# Autodesk Inventor assembly: link9_SubAssembly.ipt
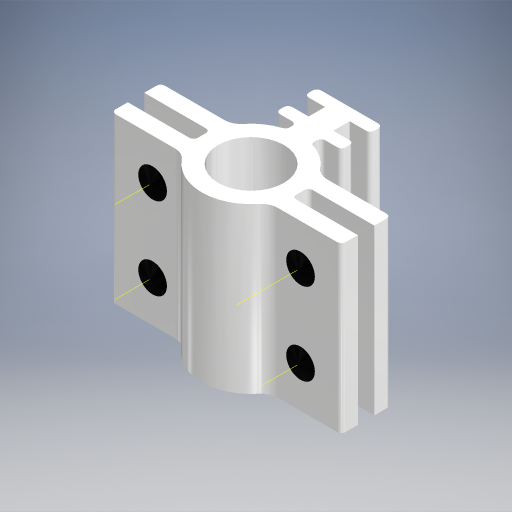
[picture p0: Inventor's stored thumbnail of the model, 512x512]
Saved by Autodesk Inventor 2024.1 (Build 281209000, 209)
## iProperties
Created: 2023-11-11
Part Number: link9_SubAssembly.ipt
Document SubType Name: Assembly
Designer: Camilo
Mass: 8.97147 g
Surface Area: 38.2594 cm^2
Volume: 3.32277 cm^3
Density: 2.7 g/cm^3
Author: Camilo
## Documents named in this file (3)
- D:\Documentos\MEGA\Universidad\2023-2\DinamicaComputacionalDeSistemasMulticuerpo\DinamicaComputacionalSistemasMulticuerpo\Proyecto\CAD\3D\link5_SubAssembly.iam
- D:\Documentos\MEGA\Universidad\2023-2\DinamicaComputacionalDeSistemasMulticuerpo\DinamicaComputacionalSistemasMulticuerpo\Proyecto\CAD\3D\link5.ipt
- D:\Documentos\MEGA\Universidad\2023-2\DinamicaComputacionalDeSistemasMulticuerpo\DinamicaComputacionalSistemasMulticuerpo\Proyecto\CAD\3D\large_bolt.ipt
## Components (5 placed, 2 different names)
1. link5:1 — Insert:1, Insert:2, Insert:3, Insert:4
2. large_bolt:1 — Insert:1
3. large_bolt:2 — Insert:2
4. large_bolt:3 — Insert:3
5. large_bolt:4 — Insert:4
## Relationships (4: Insert 4)
- Insert:1: link5:1 ↔ large_bolt:1
- Insert:2: link5:1 ↔ large_bolt:2
- Insert:3: link5:1 ↔ large_bolt:3
- Insert:4: link5:1 ↔ large_bolt:4
